# Autodesk Inventor assembly: brush holder assy v5
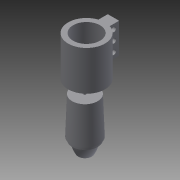
[picture p0: Inventor's stored thumbnail of the model, 180x180]
Saved by Autodesk Inventor 2013 SP2 (Build 170200200, 200)
## iProperties
Created: 2017-08-28
Part Number: brush holder assy v5
Document SubType Name: Assembly
Designer: hdv
Author: hdv
## Documents named in this file (4)
- C:\Users\hdv\Dropbox\Projects\Inventor\PaintBot_3\Brush holder\brush holder assy v5.iam
- C:\Users\hdv\Dropbox\Projects\Inventor\PaintBot_3\Brush holder\brush holder v5.ipt
- C:\Users\hdv\Dropbox\Projects\Inventor\PaintBot_3\Brush holder\brush fitting parta v5.ipt
- C:\Users\hdv\Dropbox\Projects\Inventor\PaintBot_3\Brush holder\brush fitting partb v5.ipt
## Components (3 placed, 3 different names)
1. brush holder v5:1
2. brush fitting parta v5:1 — Mate:3, Mate:4
3. brush fitting partb v5:1 — Mate:3, Mate:4
## Relationships (2: Mate 2)
- Mate:3: brush fitting parta v5:1 ↔ brush fitting partb v5:1
- Mate:4: brush fitting parta v5:1 ↔ brush fitting partb v5:1
